# Autodesk Inventor assembly: finalvideobot
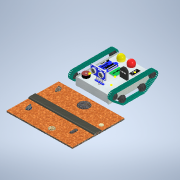
[picture p0: Inventor's stored thumbnail of the model, 180x180]
Saved by Autodesk Inventor 2021 (Build 250183000, 183)
## iProperties
Created: 2021-07-27
Part Number: finalvideobot
Document SubType Name: Assembly
Designer: preet
Author: preet
## Documents named in this file (14)
- D:\Engg Expl\Assembly\finalvideobot.iam
- D:\Engg Expl\Assembly\Chassi.ipt
- D:\Engg Expl\Assembly\tank tread.iam
- D:\Engg Expl\Assembly\arduino now.ipt
- D:\Engg Expl\Assembly\red led now.ipt
- D:\Engg Expl\Assembly\yellow led now.ipt
- D:\Engg Expl\Assembly\buzzer now.ipt
- D:\Engg Expl\Assembly\micro now.ipt
- D:\Engg Expl\Assembly\tilt now.ipt
- D:\Engg Expl\Assembly\tmp 36 now.ipt
- D:\Engg Expl\Assembly\ultrasonic now.ipt
- D:\Engg Expl\Assembly\drive motor.ipt
- D:\Engg Expl\Assembly\DC motor now.ipt
- D:\Engg Expl\Assembly\Obstacle.ipt
## Components (17 placed, 13 different names)
1. Chassi:1 — Mate:1, Mate:2, Mate:3, Mate:4, Mate:5, Mate:6, Mate:7, Mate:8, Mate:9, Mate:10, Mate:14, Mate:15, Mate:16, Mate:17
2. tank tread:1 [sub-assembly] — Mate:1, Mate:3, Mate:4, Mate:5, Mate:6, Mate:7, Mate:8, Mate:20, Mate:22
3. tank tread:2 [sub-assembly] — Mate:2, Mate:9, Tangent:1, Mate:19, Mate:21
4. arduino now:1 — Mate:10
5. buzzer now:1 — Mate:14, Tangent:1
6. micro now:1 — Mate:15, Mate:18
7. tilt now:1 — Mate:16
8. tmp 36 now:1 — Mate:17
9. ultrasonic now:1 — Mate:18
10. drive motor:1
11. DC motor now:1 — Mate:19
12. DC motor now:2 — Mate:21
13. DC motor now:3 — Mate:20
14. DC motor now:4 — Mate:22
15. yellow led now:1
16. red led now:1
17. Obstacle:1
## Relationships (20: Mate 19, Tangent 1)
- Mate:1: Chassi:1 ↔ tank tread:1
- Mate:2: Chassi:1 ↔ tank tread:2
- Mate:3: Chassi:1 ↔ tank tread:1
- Mate:4: Chassi:1 ↔ tank tread:1
- Mate:5: Chassi:1 ↔ tank tread:1
- Mate:6: Chassi:1 ↔ tank tread:1
- Mate:7: Chassi:1 ↔ tank tread:1
- Mate:8: Chassi:1 ↔ tank tread:1
- Mate:9: Chassi:1 ↔ tank tread:2
- Mate:10 (-10 mm): Chassi:1 ↔ arduino now:1
- Mate:14 (-14 mm): Chassi:1 ↔ buzzer now:1
- Mate:15 (-52 mm): Chassi:1 ↔ micro now:1
- Mate:16 (-15 mm): Chassi:1 ↔ tilt now:1
- Mate:17 (-20 mm): Chassi:1 ↔ tmp 36 now:1
- Mate:18: micro now:1 ↔ ultrasonic now:1
- Tangent:1: tank tread:2 ↔ buzzer now:1
- Mate:19 (-90 mm): tank tread:2 ↔ DC motor now:1
- Mate:20 (-90 mm): tank tread:1 ↔ DC motor now:3
- Mate:21 (-90 mm): tank tread:2 ↔ DC motor now:2
- Mate:22 (-90 mm): tank tread:1 ↔ DC motor now:4
